# Autodesk Inventor assembly: Hand
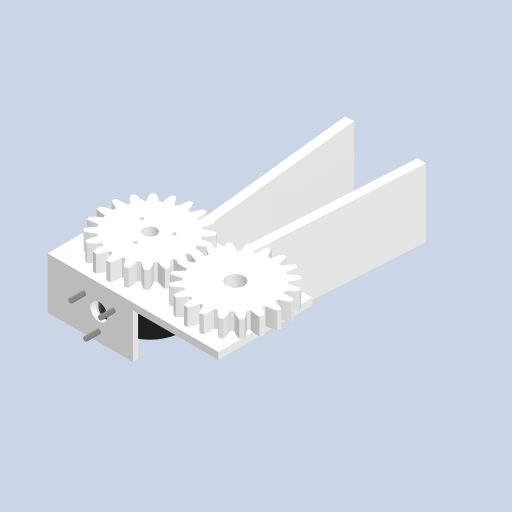
[picture p0: Inventor's stored thumbnail of the model, 512x512]
Saved by Autodesk Inventor 2023 (Build 270158000, 158)
## iProperties
Created: 2024-11-08
Part Number: Hand
Document SubType Name: Assembly
Designer: kiyo
Mass: 143.72 g
Surface Area: 584.434 cm^2
Volume: 137.311 cm^3
Density: 1.04668 g/cm^3
Author: kiyo
## Documents named in this file (11)
- D:\GitHub\inventor\syu-si\OfficeRobot\Manipulator\Hand.iam
- D:\GitHub\inventor\syu-si\OfficeRobot\Manipulator\hand-nail-1.ipt
- D:\GitHub\inventor\syu-si\OfficeRobot\Manipulator\hand-nail-2.ipt
- D:\GitHub\inventor\syu-si\OfficeRobot\ReadyMade\Screw\D3040-7130B.ipt
- D:\GitHub\inventor\syu-si\OfficeRobot\ReadyMade\Screw\D4050-9120B.ipt
- D:\GitHub\inventor\syu-si\OfficeRobot\ReadyMade\Screw\FB-305530.ipt
- D:\GitHub\inventor\syu-si\OfficeRobot\Manipulator\hand-gearbox.ipt
- D:\GitHub\inventor\syu-si\OfficeRobot\ReadyMade\Steadywin\GIM3505-8_with-driver.ipt
- D:\GitHub\inventor\syu-si\OfficeRobot\ReadyMade\Screw\FWSJJ-D5-V2_6-T4_5.ipt
- D:\GitHub\inventor\syu-si\OfficeRobot\ReadyMade\Screw\CBSST2_5-6.ipt
- D:\GitHub\inventor\syu-si\OfficeRobot\ReadyMade\Screw\M2-5_10mm.ipt
## Components (16 placed, 10 different names)
1. 平歯車1:1 — 挿入:5, 挿入:6, 挿入:7, 挿入:13
2. 平歯車2:1 — 挿入:2
3. D3040-7130B:1 — 挿入:1, 挿入:9
4. D4050-9120B:1 — 挿入:1, 挿入:2
5. FB-305530:1 — 挿入:8, 挿入:9
6. hand-gearbox:1 — 挿入:3, 挿入:4, 挿入:8, 挿入:10, 挿入:11, 挿入:12, 挿入:14, 挿入:15, 挿入:16
7. GIM3505-8_with-driver:1 — 挿入:3, 挿入:4, 挿入:13
8. FWSJJ-D5-V2_6-T4_5:1 — 挿入:5
9. FWSJJ-D5-V2_6-T4_5:2 — 挿入:6
10. FWSJJ-D5-V2_6-T4_5:3 — 挿入:7
11. CBSST2_5-6:1 — 挿入:12
12. CBSST2_5-6:2 — 挿入:11
13. CBSST2_5-6:3 — 挿入:10
14. M2-5_10mm:1 — 挿入:14
15. M2-5_10mm:2 — 挿入:15
16. M2-5_10mm:3 — 挿入:16
## Relationships (16: Insert 16)
- 挿入:1 [Insert]: D3040-7130B:1 ↔ D4050-9120B:1
- 挿入:2 [Insert]: 平歯車2:1 ↔ D4050-9120B:1
- 挿入:3 [Insert]: hand-gearbox:1 ↔ GIM3505-8_with-driver:1
- 挿入:4 [Insert]: hand-gearbox:1 ↔ GIM3505-8_with-driver:1
- 挿入:5 [Insert]: 平歯車1:1 ↔ FWSJJ-D5-V2_6-T4_5:1
- 挿入:6 [Insert]: 平歯車1:1 ↔ FWSJJ-D5-V2_6-T4_5:2
- 挿入:7 [Insert]: 平歯車1:1 ↔ FWSJJ-D5-V2_6-T4_5:3
- 挿入:8 [Insert]: FB-305530:1 ↔ hand-gearbox:1
- 挿入:9 [Insert]: D3040-7130B:1 ↔ FB-305530:1
- 挿入:10 [Insert]: hand-gearbox:1 ↔ CBSST2_5-6:3
- 挿入:11 [Insert]: hand-gearbox:1 ↔ CBSST2_5-6:2
- 挿入:12 [Insert]: hand-gearbox:1 ↔ CBSST2_5-6:1
- 挿入:13 [Insert] (4 mm): 平歯車1:1 ↔ GIM3505-8_with-driver:1
- 挿入:14 [Insert]: hand-gearbox:1 ↔ M2-5_10mm:1
- 挿入:15 [Insert]: hand-gearbox:1 ↔ M2-5_10mm:2
- 挿入:16 [Insert]: hand-gearbox:1 ↔ M2-5_10mm:3
